# Autodesk Inventor assembly: Pancake_Timing Assy_Lever Shaft 2
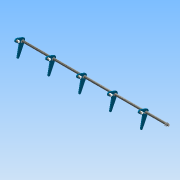
[picture p0: Inventor's stored thumbnail of the model, 180x180]
Saved by Autodesk Inventor 2018.1 (Build 221171000, 171)
## iProperties
Created: 2019-02-11
Part Number: Pancake_Timing Assy_Lever Shaft 2
Document SubType Name: Assembly
Designer: James
Author: James
## Documents named in this file (7)
- C:\Users\admin\Desktop\Ball Sorting Machine\Ball-Sorting-Machine\Pancake Sort\Pancake_Timing Assy_Lever Shaft 2.iam
- C:\Users\admin\Desktop\Ball Sorting Machine\Ball-Sorting-Machine\Prototype CAD\Selection Sort - 40mm\BS 3673 - 6mm External Circlip.ipt
- C:\Users\admin\Desktop\Ball Sorting Machine\Ball-Sorting-Machine\Timing Gate\M3 x 0.5mm Zinc Plated Steel Washer.ipt
- C:\Users\admin\Desktop\Ball Sorting Machine\Ball-Sorting-Machine\Timing Gate\Socket Button Head - (A2) - M3 x 10.ipt
- C:\Users\admin\Desktop\Ball Sorting Machine\Ball-Sorting-Machine\Timing Gate\Timing_Lever Weight.ipt
- C:\Users\admin\Desktop\Ball Sorting Machine\Ball-Sorting-Machine\Pancake Sort\Pancake_Lever Shaft 2.ipt
- C:\Users\admin\Desktop\Ball Sorting Machine\Ball-Sorting-Machine\Pancake Sort\Pancake_Lever.ipt
## Components (33 placed, 6 different names)
1. Pancake_Lever Shaft 2:1 — Mate:45, Flush:18, Mate:46, Mate:47, Mate:48, Mate:49, Mate:52, Mate:53, Mate:54, Mate:55
2. BS 3673 - 6mm External Circlip:11 — Mate:52, Mate:55, Flush:20, Flush:21
3. BS 3673 - 6mm External Circlip:12 — Mate:53, Mate:54, Flush:20
4. BS 3673 - 6mm External Circlip:1 — Flush:10, Mate:46, Mate:49, Flush:19, Angle:3
5. Pancake_Lever:1 — Mate:13, Mate:14, Mate:16, Mate:45, Flush:18, Mate:51
6. BS 3673 - 6mm External Circlip:2 — Flush:10, Angle:2, Mate:47, Mate:48, Flush:19
7. Socket Button Head - (A2) - M3 x 10:1 — Mate:15, Mate:16, Mate:50
8. M3 x 0.5mm Zinc Plated Steel Washer:1 — Mate:13, Mate:14, Mate:15
9. Timing_Lever Weight:1 — Mate:50, Mate:51
10. BS 3673 - 6mm External Circlip:3
11. Pancake_Lever:2
12. BS 3673 - 6mm External Circlip:4
13. Socket Button Head - (A2) - M3 x 10:2
14. M3 x 0.5mm Zinc Plated Steel Washer:2
15. Timing_Lever Weight:2
16. BS 3673 - 6mm External Circlip:5
17. Pancake_Lever:3
18. BS 3673 - 6mm External Circlip:6
19. Socket Button Head - (A2) - M3 x 10:3
20. M3 x 0.5mm Zinc Plated Steel Washer:3
21. Timing_Lever Weight:3
22. BS 3673 - 6mm External Circlip:7
23. Pancake_Lever:4
24. BS 3673 - 6mm External Circlip:8
25. Socket Button Head - (A2) - M3 x 10:4
26. M3 x 0.5mm Zinc Plated Steel Washer:4
27. Timing_Lever Weight:4
28. BS 3673 - 6mm External Circlip:9 — Flush:21
29. Pancake_Lever:5
30. BS 3673 - 6mm External Circlip:10
31. Socket Button Head - (A2) - M3 x 10:5
32. M3 x 0.5mm Zinc Plated Steel Washer:5
33. Timing_Lever Weight:5
## Component patterns: (5 elements, first: BS 3673 - 6mm External Circlip:1 + Pancake_Lever:1 + BS 3673 - 6mm External Circlip:2 + Socket Button Head - (A2) - M3 x 10:1 + M3 x 0.5mm Zinc Plated Steel Washer:1 + Timing_Lever Weight:1)
## Relationships (28: Mate 15, Flush 11, Angle 2)
- [Flush]: Pancake_Lever Shaft 2:1
- Flush:10: BS 3673 - 6mm External Circlip:1 ↔ BS 3673 - 6mm External Circlip:2
- Angle:2 (180 deg): BS 3673 - 6mm External Circlip:2
- Mate:13: Pancake_Lever:1 ↔ M3 x 0.5mm Zinc Plated Steel Washer:1
- Mate:14: Pancake_Lever:1 ↔ M3 x 0.5mm Zinc Plated Steel Washer:1
- Mate:15: Socket Button Head - (A2) - M3 x 10:1 ↔ M3 x 0.5mm Zinc Plated Steel Washer:1
- Mate:16: Pancake_Lever:1 ↔ Socket Button Head - (A2) - M3 x 10:1
- Flush:11 (-58 mm)
- Flush:12 (-5 mm)
- Flush:13 (30 mm)
- [Flush]: Pancake_Lever Shaft 2:1
- [Flush]: Pancake_Lever Shaft 2:1
- Mate:45: Pancake_Lever Shaft 2:1 ↔ Pancake_Lever:1
- Flush:18: Pancake_Lever Shaft 2:1 ↔ Pancake_Lever:1
- Mate:46: Pancake_Lever Shaft 2:1 ↔ BS 3673 - 6mm External Circlip:1
- Mate:47: Pancake_Lever Shaft 2:1 ↔ BS 3673 - 6mm External Circlip:2
- Mate:48: Pancake_Lever Shaft 2:1 ↔ BS 3673 - 6mm External Circlip:2
- Mate:49: Pancake_Lever Shaft 2:1 ↔ BS 3673 - 6mm External Circlip:1
- Flush:19: BS 3673 - 6mm External Circlip:1 ↔ BS 3673 - 6mm External Circlip:2
- Angle:3 (0 deg): BS 3673 - 6mm External Circlip:1
- Mate:50: Socket Button Head - (A2) - M3 x 10:1 ↔ Timing_Lever Weight:1
- Mate:51: Pancake_Lever:1 ↔ Timing_Lever Weight:1
- Mate:52: Pancake_Lever Shaft 2:1 ↔ BS 3673 - 6mm External Circlip:11
- Mate:53: Pancake_Lever Shaft 2:1 ↔ BS 3673 - 6mm External Circlip:12
- Mate:54: Pancake_Lever Shaft 2:1 ↔ BS 3673 - 6mm External Circlip:12
- Mate:55: Pancake_Lever Shaft 2:1 ↔ BS 3673 - 6mm External Circlip:11
- Flush:20: BS 3673 - 6mm External Circlip:11 ↔ BS 3673 - 6mm External Circlip:12
- Flush:21: BS 3673 - 6mm External Circlip:11 ↔ BS 3673 - 6mm External Circlip:9
